# Autodesk Inventor assembly: CIM_MotorHub_4_inch_wheel
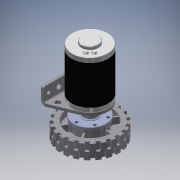
[picture p0: Inventor's stored thumbnail of the model, 180x180]
Saved by Autodesk Inventor 2016 SP1 (Build 200210100, 210)
## iProperties
Created: 2016-02-07
Part Number: CIM_MotorHub_4_inch_wheel
Document SubType Name: Assembly
Designer: steele
Author: steele
## Documents named in this file (5)
- C:\snobotics\CAD-Development\robSteele\SnoBotics2016\2016-05-05-ShooterPrototype\CIM_MotorHub_4_inch_wheel.iam
- C:\snobotics\CAD-Development\robSteele\SnoBotics2016\AM Parts\4 in HiGrip Wheel.iam
- C:\snobotics\CAD-Development\robSteele\SnoBotics2016\AM Parts\am-0320a_8mm_Key_Hub.ipt
- C:\snobotics\CAD-Development\robSteele\SnoBotics2016\AM Parts\AM 2488 CIM bracket.ipt
- C:\snobotics\CAD-Development\robSteele\SnoBotics2016\VexParts\MOT_MiniCIMMotor_217-3371.ipt
## Components (4 placed, 4 different names)
1. 4 in HiGrip Wheel:2 [sub-assembly] — Insert:1
2. am-0320a_8mm_Key_Hub:1 — Insert:1, Insert:3
3. MOT_MiniCIMMotor_217-3371:1 — Insert:4
4. AM 2488 CIM bracket:1 — Insert:3, Insert:4
## Relationships (3: Insert 3)
- Insert:1: 4 in HiGrip Wheel:2 ↔ am-0320a_8mm_Key_Hub:1
- Insert:3: am-0320a_8mm_Key_Hub:1 ↔ AM 2488 CIM bracket:1
- Insert:4: MOT_MiniCIMMotor_217-3371:1 ↔ AM 2488 CIM bracket:1
